# Autodesk Inventor assembly: nema 17 with extended mount
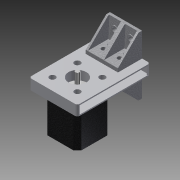
[picture p0: Inventor's stored thumbnail of the model, 180x180]
Saved by Autodesk Inventor 2015 (Build 190159000, 159)
## iProperties
Created: 2013-08-04
Part Number: nema 17 with extended mount
Document SubType Name: Assembly
Designer: mhgreen
Author: mhgreen
## Documents named in this file (4)
- C:\Users\Michael\Dropbox\autocad\openbuild\nema 17 with extended mount.iam
- C:\Users\Michael\Dropbox\autocad\openbuild\parts\NEMA17-mount-extended-plastic.ipt
- C:\Users\Michael\Dropbox\autocad\openbuild\parts\HBLFSN5hblfsn5.ipt
- C:\Users\Michael\Dropbox\autocad\openbuild\parts\NEMA17-dual-shaft.ipt
## Components (6 placed, 3 different names)
1. NEMA17-mount-extended-plastic:1 — Insert:1, Flush:1, Flush:2, Insert:2, Insert:3, Insert:4, Insert:5, Flush:3, Flush:4
2. HBLFSN5hblfsn5:1 — Insert:1, Flush:1
3. HBLFSN5hblfsn5:2 — Flush:2, Insert:2
4. NEMA17-dual-shaft:1 — Insert:3
5. HBLFSN5hblfsn5:3 — Insert:5, Flush:4
6. HBLFSN5hblfsn5:4 — Insert:4, Flush:3
## Relationships (9: Insert 5, Flush 4)
- Insert:1: NEMA17-mount-extended-plastic:1 ↔ HBLFSN5hblfsn5:1
- Flush:1: NEMA17-mount-extended-plastic:1 ↔ HBLFSN5hblfsn5:1
- Flush:2: NEMA17-mount-extended-plastic:1 ↔ HBLFSN5hblfsn5:2
- Insert:2: NEMA17-mount-extended-plastic:1 ↔ HBLFSN5hblfsn5:2
- Insert:3: NEMA17-mount-extended-plastic:1 ↔ NEMA17-dual-shaft:1
- Insert:4: NEMA17-mount-extended-plastic:1 ↔ HBLFSN5hblfsn5:4
- Insert:5: NEMA17-mount-extended-plastic:1 ↔ HBLFSN5hblfsn5:3
- Flush:3: NEMA17-mount-extended-plastic:1 ↔ HBLFSN5hblfsn5:4
- Flush:4: NEMA17-mount-extended-plastic:1 ↔ HBLFSN5hblfsn5:3
